# Autodesk Inventor assembly: 3-10
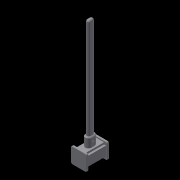
[picture p0: Inventor's stored thumbnail of the model, 180x180]
Saved by Autodesk Inventor 2017 (Build 210142000, 142)
## iProperties
Part Number: 3-10
Material: 一般
Document SubType Name: Assembly
Designer: r0909
Author: r0909
## Documents named in this file (5)
- C:\Users\r0909\Desktop\inventor\3-10.iam
- C:\Users\r0909\Desktop\inventor\3-6.ipt
- C:\Users\r0909\Desktop\inventor\3-7.ipt
- C:\Users\r0909\Desktop\inventor\3-8.ipt
- C:\Users\r0909\Desktop\inventor\3-10.1.ipt
## Components (8 placed, 4 different names)
1. 3-6:1 — 貼合:1, 角度:1, 齊平:1, 角度:2, 齊平:4, 貼合:3, 齊平:7, 齊平:8, 貼合:9
2. 3-7:1 — 貼合:1, 角度:1, 齊平:1, 齊平:2, 齊平:3, 貼合:2, 齊平:4, 齊平:5, 貼合:4, 齊平:6, 貼合:7, 貼合:10, 貼合:11, 相切:1
3. 3-8:1 — 貼合:9, 貼合:10, 貼合:11, 貼合:12, 貼合:13
4. 3-7:2 — 齊平:2, 角度:2, 齊平:3, 貼合:2, 貼合:5, 貼合:6
5. 3-7:3 — 貼合:3, 齊平:5, 貼合:4, 貼合:5, 貼合:8
6. 3-7:4 — 齊平:6, 貼合:6, 貼合:7
7. 3-6:2 — 貼合:8, 齊平:7, 齊平:8
8. 3-10.1:1 — 貼合:12, 貼合:13, 相切:1
## Relationships (24: Mate 13, Flush 8, Angle 2, Tangent 1)
- 貼合:1 [Mate]: 3-6:1 ↔ 3-7:1
- 角度:1 [Angle] (0 deg): 3-6:1 ↔ 3-7:1
- 齊平:1 [Flush] (8 mm): 3-6:1 ↔ 3-7:1
- 齊平:2 [Flush]: 3-7:1 ↔ 3-7:2
- 角度:2 [Angle] (0 deg): 3-6:1 ↔ 3-7:2
- 齊平:3 [Flush]: 3-7:1 ↔ 3-7:2
- 貼合:2 [Mate] (60 mm): 3-7:1 ↔ 3-7:2
- 齊平:4 [Flush]: 3-6:1 ↔ 3-7:1
- 貼合:3 [Mate]: 3-6:1 ↔ 3-7:3
- 齊平:5 [Flush]: 3-7:1 ↔ 3-7:3
- 貼合:4 [Mate]: 3-7:1 ↔ 3-7:3
- 貼合:5 [Mate]: 3-7:2 ↔ 3-7:3
- 齊平:6 [Flush]: 3-7:1 ↔ 3-7:4
- 貼合:6 [Mate]: 3-7:2 ↔ 3-7:4
- 貼合:7 [Mate]: 3-7:1 ↔ 3-7:4
- 貼合:8 [Mate]: 3-7:3 ↔ 3-6:2
- 齊平:7 [Flush]: 3-6:1 ↔ 3-6:2
- 齊平:8 [Flush]: 3-6:1 ↔ 3-6:2
- 貼合:9 [Mate] (60 mm): 3-6:1 ↔ 3-8:1
- 貼合:10 [Mate]: 3-7:1 ↔ 3-8:1
- 貼合:11 [Mate]: 3-7:1 ↔ 3-8:1
- 貼合:12 [Mate]: 3-8:1 ↔ 3-10.1:1
- 貼合:13 [Mate]: 3-8:1 ↔ 3-10.1:1
- 相切:1 [Tangent]: 3-7:1 ↔ 3-10.1:1
